# Autodesk Inventor assembly: Ballscrew_Assembly_1204
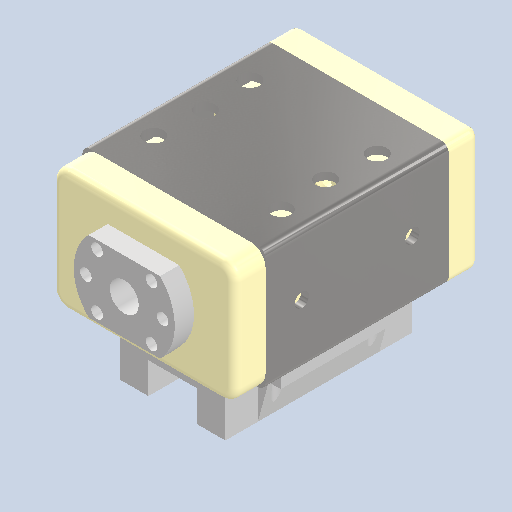
[picture p0: Inventor's stored thumbnail of the model, 512x512]
Saved by Autodesk Inventor 2023 (Build 270158000, 158)
## iProperties
Created: 2022-05-04
Part Number: Ballscrew_Assembly_1204
Document SubType Name: Assembly
Designer: plebbb
Author: plebbb
## Documents named in this file (6)
- C:\Users\think\OneDrive\Desktop\CNC_Project\Ballscrew_Assembly_1204.iam
- C:\Users\think\OneDrive\Desktop\CNC_Project\2x3_Spacer_1204_Rear.ipt
- C:\Users\think\OneDrive\Desktop\CNC_Project\2x3_Spacer_1204.ipt
- C:\Users\think\OneDrive\Desktop\CNC_Project\SFU1204_Nut.ipt
- C:\Users\think\OneDrive\Desktop\CNC_Project\2x3_Tube_Short.ipt
- C:\Users\think\OneDrive\Desktop\CNC_Project\HGW20CC_Slider.ipt
## Components (5 placed, 5 different names)
1. 2x3_Spacer_1204_Rear:1
2. 2x3_Spacer_1204:1
3. SFU1204_Nut:1
4. 2x3_Tube_Short:1
5. HGW20CC_Slider:1
## Relationships (12: Mate 8, Flush 4)
- [Flush]: 2x3_Spacer_1204:1 ↔ 2x3_Tube_Short:1
- [Flush]: 2x3_Spacer_1204:1 ↔ 2x3_Tube_Short:1
- [Mate]: 2x3_Spacer_1204:1 ↔ 2x3_Tube_Short:1
- [Flush]: 2x3_Spacer_1204_Rear:1 ↔ 2x3_Tube_Short:1
- [Flush]: 2x3_Spacer_1204_Rear:1 ↔ 2x3_Tube_Short:1
- [Mate]: 2x3_Spacer_1204_Rear:1 ↔ 2x3_Tube_Short:1
- [Mate]: 2x3_Spacer_1204:1 ↔ SFU1204_Nut:1
- [Mate]: 2x3_Spacer_1204:1 ↔ SFU1204_Nut:1
- [Mate]: 2x3_Spacer_1204:1 ↔ SFU1204_Nut:1
- [Mate]: 2x3_Tube_Short:1 ↔ HGW20CC_Slider:1
- [Mate]: 2x3_Tube_Short:1 ↔ HGW20CC_Slider:1
- [Mate]: 2x3_Tube_Short:1 ↔ HGW20CC_Slider:1
